# Autodesk Inventor assembly: GE-13021
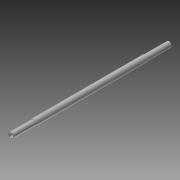
[picture p0: Inventor's stored thumbnail of the model, 180x180]
Saved by Autodesk Inventor 2013 (Build 170138000, 138)
## iProperties
Created: 2013-01-06
Part Number: GE-13021
Document SubType Name: Assembly
Designer: Phillip
Author: Phillip
## Documents named in this file (3)
- E:\Data Folder\FIRST 2013\FIRST KOP\FIRST Arena 2013\Pyramid\GE-13021.iam
- E:\Data Folder\FIRST 2013\FIRST KOP\FIRST Arena 2013\Pyramid\GE-13021-01.ipt
- E:\Data Folder\FIRST 2013\FIRST KOP\FIRST Arena 2013\Pyramid\GE-13021-02.ipt
## Components (3 placed, 2 different names)
1. GE-13021-01:1 — Insert:1, Insert:2
2. GE-13021-02:1 — Insert:1
3. GE-13021-02:2 — Insert:2
## Relationships (2: Insert 2)
- Insert:1 (-146.05 mm): GE-13021-01:1 ↔ GE-13021-02:1
- Insert:2 (-146.05 mm): GE-13021-01:1 ↔ GE-13021-02:2
